# Autodesk Inventor assembly: Base2
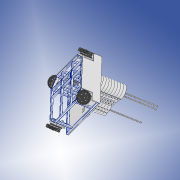
[picture p0: Inventor's stored thumbnail of the model, 180x180]
Saved by Autodesk Inventor 2017 SP1 (Build 210196100, 196)
## iProperties
Created: 2017-06-13
Part Number: Base2
Document SubType Name: Assembly
Designer: zallen
Author: zallen
## Documents named in this file (10)
- C:\Users\Zach\Documents\GitHub\cr-laundry-robot\src\Base\Base.iam
- C:\Users\Zach\Documents\GitHub\cr-laundry-robot\src\Base\Chassis\Chassis.iam
- C:\Users\Zach\Documents\GitHub\cr-laundry-robot\lib\Linear Actuator 450mm\LinearActuator450mm.iam
- C:\Users\Zach\Documents\GitHub\cr-laundry-robot\src\Base\Top Cover.ipt
- C:\Users\Zach\Documents\GitHub\cr-laundry-robot\src\Base\Front Cover.ipt
- C:\Users\Zach\Documents\GitHub\cr-laundry-robot\src\Base\Wheel Assembly\Wheel Assembly.iam
- C:\Users\Zach\Documents\GitHub\cr-laundry-robot\src\Base\Riser Base - Center.ipt
- C:\Users\Zach\Documents\GitHub\cr-laundry-robot\src\Base\Riser Base - Outer.ipt
- C:\Users\Zach\Documents\GitHub\cr-laundry-robot\src\Base\Quick Shaft 12mm x 500mm.ipt
- C:\Users\Zach\Documents\GitHub\cr-laundry-robot\src\Base\Rod End Stop.ipt
## Components (57 placed, 9 different names)
1. Chassis:1 [sub-assembly] — Mate:17, Mate:23, Mate:25, Mate:28, Mate:29, Mate:30, Mate:33, Mate:36, Mate:37, Mate:38, Mate:39, Mate:40, Mate:41, Mate:42, Mate:43, Mate:44, Mate:45, Mate:46, Mate:47, Mate:48, Mate:49, Mate:50, Mate:51, Mate:53, Mate:55
2. LinearActuator450mm:1 [sub-assembly] — Mate:17
3. Top Cover:1 — Mate:23, Mate:24, Mate:26, Mate:27, Mate:31, Mate:32, Mate:34, Mate:52, Mate:54, Mate:57, Mate:159, Mate:161
4. Front Cover:1 — Mate:24, Mate:25, Mate:26, Mate:35
5. Front Cover:2 — Mate:27, Mate:28, Mate:29
6. Front Cover:3 — Mate:33, Mate:34, Mate:35
7. Front Cover:4 — Mate:30, Mate:31, Mate:32
8. Wheel Assembly:1 [sub-assembly] — Mate:36, Mate:37, Mate:38, Mate:39, Mate:40
9. Wheel Assembly:2 [sub-assembly] — Mate:41, Mate:42, Mate:43
10. Wheel Assembly:3 [sub-assembly] — Mate:44, Mate:45, Mate:46
11. Wheel Assembly:4 [sub-assembly] — Mate:47, Mate:48, Mate:49
12. Riser Base - Center:1 — Mate:50, Mate:51, Mate:52, Flush:60, Mate:58, Mate:137, Mate:138
13. Riser Base - Center:2 — Mate:53, Mate:54, Mate:55, Mate:56, Flush:58, Flush:59, Flush:61, Mate:119
14. Riser Base - Outer:1 — Mate:56, Flush:58, Flush:59, Mate:86, Mate:87, Mate:88
15. Riser Base - Outer:2 — Flush:60, Mate:57, Mate:58, Mate:59, Mate:60, Mate:61
16. Riser Base - Outer:3 — Mate:59, Mate:60, Mate:61, Mate:62, Mate:63, Mate:64
17. Riser Base - Outer:4 — Mate:68, Mate:69, Mate:70, Mate:71, Mate:72, Mate:73
18. Riser Base - Outer:5 — Mate:65, Mate:66, Mate:67, Mate:68, Mate:69, Mate:70
19. Riser Base - Outer:6 — Mate:62, Mate:63, Mate:64, Mate:65, Mate:66, Mate:67
20. Riser Base - Outer:7 — Mate:74, Mate:75, Mate:76, Mate:77, Mate:78, Mate:79
21. Riser Base - Outer:8 — Mate:80, Mate:81, Mate:82, Mate:83, Mate:84, Mate:85
22. Riser Base - Outer:9 — Mate:83, Mate:84, Mate:85, Mate:157
23. Riser Base - Outer:10 — Mate:77, Mate:78, Mate:79, Mate:80, Mate:81, Mate:82
24. Riser Base - Outer:11 — Mate:71, Mate:72, Mate:73, Mate:74, Mate:75, Mate:76
25. Riser Base - Outer:12 — Mate:86, Mate:87, Mate:88, Mate:89, Mate:90, Mate:91
26. Riser Base - Outer:13 — Mate:92, Mate:93, Mate:94, Mate:95, Mate:96, Mate:97
27. Riser Base - Outer:14 — Mate:98, Mate:99, Mate:100, Mate:101, Mate:102, Mate:104, Mate:105, Mate:106
28. Riser Base - Outer:15 — Mate:107, Mate:108, Mate:109, Mate:110, Mate:111, Mate:112, Mate:115
29. Riser Base - Outer:16 — Mate:113, Mate:114, Mate:115
30. Riser Base - Outer:17 — Mate:110, Mate:111, Mate:112, Mate:113, Mate:114, Mate:116, Mate:117, Mate:118
31. Riser Base - Outer:18 — Mate:95, Mate:96, Mate:97, Mate:98, Mate:99, Mate:100, Mate:103
32. Riser Base - Outer:19 — Mate:89, Mate:90, Mate:91, Mate:92, Mate:93, Mate:94
33. Riser Base - Outer:20 — Mate:101, Mate:102, Mate:103
34. Riser Base - Outer:21 — Mate:104, Mate:105, Mate:106, Mate:107, Mate:108, Mate:109
35. Riser Base - Outer:22 — Mate:116, Mate:117, Mate:118, Mate:155, Mate:158
36. Riser Base - Center:3 — Mate:120, Mate:121, Mate:122, Mate:123, Mate:124
37. Riser Base - Center:4 — Flush:61, Mate:119, Mate:120, Mate:121
38. Riser Base - Center:5 — Mate:122, Mate:123, Mate:124, Mate:125, Mate:126
39. Riser Base - Center:6 — Mate:129, Mate:130, Mate:131, Mate:132
40. Riser Base - Center:7 — Mate:127, Mate:128, Mate:129, Mate:130
41. Riser Base - Center:8 — Mate:125, Mate:126, Mate:127, Mate:128
42. Riser Base - Center:9 — Mate:131, Mate:132, Mate:133, Mate:134
43. Riser Base - Center:10 — Mate:133, Mate:134, Mate:135, Mate:136
44. Riser Base - Center:11 — Mate:135, Mate:136, Mate:155
45. Riser Base - Center:12 — Mate:137, Mate:138, Mate:139, Mate:140
46. Riser Base - Center:13 — Mate:139, Mate:140, Mate:141, Mate:142
47. Riser Base - Center:14 — Mate:141, Mate:142, Mate:143, Mate:144
48. Riser Base - Center:15 — Mate:143, Mate:144, Mate:145, Mate:146
49. Riser Base - Center:16 — Mate:145, Mate:146, Mate:147, Mate:148
50. Riser Base - Center:17 — Mate:147, Mate:148, Mate:149, Mate:150
51. Riser Base - Center:18 — Mate:149, Mate:150, Mate:151, Mate:152
52. Riser Base - Center:19 — Mate:151, Mate:152, Mate:153, Mate:154
53. Riser Base - Center:20 — Mate:153, Mate:154, Mate:160, Mate:162
54. Quick Shaft 12mm x 500mm:1 — Mate:157, Flush:62, Mate:159
55. Quick Shaft 12mm x 500mm:2 — Mate:158, Flush:62
56. Quick Shaft 12mm x 500mm:3 — Mate:162, Mate:163
57. Rod End Stop:1 — Mate:160, Mate:161, Mate:163
## Relationships (146: Mate 141, Flush 5)
- Mate:17: Chassis:1 ↔ LinearActuator450mm:1
- Mate:23: Chassis:1 ↔ Top Cover:1
- Mate:24: Top Cover:1 ↔ Front Cover:1
- Mate:25: Chassis:1 ↔ Front Cover:1
- Mate:26: Top Cover:1 ↔ Front Cover:1
- Mate:27: Top Cover:1 ↔ Front Cover:2
- Mate:28: Chassis:1 ↔ Front Cover:2
- Mate:29: Chassis:1 ↔ Front Cover:2
- Mate:30: Chassis:1 ↔ Front Cover:4
- Mate:31: Top Cover:1 ↔ Front Cover:4
- Mate:32: Top Cover:1 ↔ Front Cover:4
- Mate:33: Chassis:1 ↔ Front Cover:3
- Mate:34: Top Cover:1 ↔ Front Cover:3
- Mate:35: Front Cover:1 ↔ Front Cover:3
- Mate:36: Chassis:1 ↔ Wheel Assembly:1
- Mate:37: Chassis:1 ↔ Wheel Assembly:1
- Mate:38: Chassis:1 ↔ Wheel Assembly:1
- Mate:39: Chassis:1 ↔ Wheel Assembly:1
- Mate:40: Chassis:1 ↔ Wheel Assembly:1
- Mate:41: Chassis:1 ↔ Wheel Assembly:2
- Mate:42: Chassis:1 ↔ Wheel Assembly:2
- Mate:43: Chassis:1 ↔ Wheel Assembly:2
- Mate:44: Chassis:1 ↔ Wheel Assembly:3
- Mate:45: Chassis:1 ↔ Wheel Assembly:3
- Mate:46: Chassis:1 ↔ Wheel Assembly:3
- Mate:47: Chassis:1 ↔ Wheel Assembly:4
- Mate:48: Chassis:1 ↔ Wheel Assembly:4
- Mate:49: Chassis:1 ↔ Wheel Assembly:4
- Mate:50: Chassis:1 ↔ Riser Base - Center:1
- Mate:51: Chassis:1 ↔ Riser Base - Center:1
- Mate:52: Top Cover:1 ↔ Riser Base - Center:1
- Mate:53: Chassis:1 ↔ Riser Base - Center:2
- Mate:54: Top Cover:1 ↔ Riser Base - Center:2
- Mate:55: Chassis:1 ↔ Riser Base - Center:2
- Mate:56: Riser Base - Center:2 ↔ Riser Base - Outer:1
- Flush:58: Riser Base - Center:2 ↔ Riser Base - Outer:1
- Flush:59: Riser Base - Center:2 ↔ Riser Base - Outer:1
- Flush:60: Riser Base - Center:1 ↔ Riser Base - Outer:2
- Mate:57: Top Cover:1 ↔ Riser Base - Outer:2
- Mate:58: Riser Base - Center:1 ↔ Riser Base - Outer:2
- Mate:59: Riser Base - Outer:2 ↔ Riser Base - Outer:3
- Mate:60: Riser Base - Outer:2 ↔ Riser Base - Outer:3
- Mate:61: Riser Base - Outer:2 ↔ Riser Base - Outer:3
- Mate:62: Riser Base - Outer:3 ↔ Riser Base - Outer:6
- Mate:63: Riser Base - Outer:3 ↔ Riser Base - Outer:6
- Mate:64: Riser Base - Outer:3 ↔ Riser Base - Outer:6
- Mate:65: Riser Base - Outer:5 ↔ Riser Base - Outer:6
- Mate:66: Riser Base - Outer:5 ↔ Riser Base - Outer:6
- Mate:67: Riser Base - Outer:5 ↔ Riser Base - Outer:6
- Mate:68: Riser Base - Outer:4 ↔ Riser Base - Outer:5
- Mate:69: Riser Base - Outer:4 ↔ Riser Base - Outer:5
- Mate:70: Riser Base - Outer:4 ↔ Riser Base - Outer:5
- Mate:71: Riser Base - Outer:4 ↔ Riser Base - Outer:11
- Mate:72: Riser Base - Outer:4 ↔ Riser Base - Outer:11
- Mate:73: Riser Base - Outer:4 ↔ Riser Base - Outer:11
- Mate:74: Riser Base - Outer:7 ↔ Riser Base - Outer:11
- Mate:75: Riser Base - Outer:7 ↔ Riser Base - Outer:11
- Mate:76: Riser Base - Outer:7 ↔ Riser Base - Outer:11
- Mate:77: Riser Base - Outer:7 ↔ Riser Base - Outer:10
- Mate:78: Riser Base - Outer:7 ↔ Riser Base - Outer:10
- Mate:79: Riser Base - Outer:7 ↔ Riser Base - Outer:10
- Mate:80: Riser Base - Outer:8 ↔ Riser Base - Outer:10
- Mate:81: Riser Base - Outer:8 ↔ Riser Base - Outer:10
- Mate:82: Riser Base - Outer:8 ↔ Riser Base - Outer:10
- Mate:83: Riser Base - Outer:8 ↔ Riser Base - Outer:9
- Mate:84: Riser Base - Outer:8 ↔ Riser Base - Outer:9
- Mate:85: Riser Base - Outer:8 ↔ Riser Base - Outer:9
- Mate:86: Riser Base - Outer:1 ↔ Riser Base - Outer:12
- Mate:87: Riser Base - Outer:1 ↔ Riser Base - Outer:12
- Mate:88: Riser Base - Outer:1 ↔ Riser Base - Outer:12
- Mate:89: Riser Base - Outer:12 ↔ Riser Base - Outer:19
- Mate:90: Riser Base - Outer:12 ↔ Riser Base - Outer:19
- Mate:91: Riser Base - Outer:12 ↔ Riser Base - Outer:19
- Mate:92: Riser Base - Outer:13 ↔ Riser Base - Outer:19
- Mate:93: Riser Base - Outer:13 ↔ Riser Base - Outer:19
- Mate:94: Riser Base - Outer:13 ↔ Riser Base - Outer:19
- Mate:95: Riser Base - Outer:13 ↔ Riser Base - Outer:18
- Mate:96: Riser Base - Outer:13 ↔ Riser Base - Outer:18
- Mate:97: Riser Base - Outer:13 ↔ Riser Base - Outer:18
- Mate:98: Riser Base - Outer:14 ↔ Riser Base - Outer:18
- Mate:99: Riser Base - Outer:14 ↔ Riser Base - Outer:18
- Mate:100: Riser Base - Outer:14 ↔ Riser Base - Outer:18
- Mate:101: Riser Base - Outer:14 ↔ Riser Base - Outer:20
- Mate:102: Riser Base - Outer:14 ↔ Riser Base - Outer:20
- Mate:103: Riser Base - Outer:18 ↔ Riser Base - Outer:20
- Mate:104: Riser Base - Outer:14 ↔ Riser Base - Outer:21
- Mate:105: Riser Base - Outer:14 ↔ Riser Base - Outer:21
- Mate:106: Riser Base - Outer:14 ↔ Riser Base - Outer:21
- Mate:107: Riser Base - Outer:15 ↔ Riser Base - Outer:21
- Mate:108: Riser Base - Outer:15 ↔ Riser Base - Outer:21
- Mate:109: Riser Base - Outer:15 ↔ Riser Base - Outer:21
- Mate:110: Riser Base - Outer:15 ↔ Riser Base - Outer:17
- Mate:111: Riser Base - Outer:15 ↔ Riser Base - Outer:17
- Mate:112: Riser Base - Outer:15 ↔ Riser Base - Outer:17
- Mate:113: Riser Base - Outer:16 ↔ Riser Base - Outer:17
- Mate:114: Riser Base - Outer:16 ↔ Riser Base - Outer:17
- Mate:115: Riser Base - Outer:15 ↔ Riser Base - Outer:16
- Mate:116: Riser Base - Outer:17 ↔ Riser Base - Outer:22
- Mate:117: Riser Base - Outer:17 ↔ Riser Base - Outer:22
- Mate:118: Riser Base - Outer:17 ↔ Riser Base - Outer:22
- Flush:61: Riser Base - Center:2 ↔ Riser Base - Center:4
- Mate:119: Riser Base - Center:2 ↔ Riser Base - Center:4
- Mate:120: Riser Base - Center:3 ↔ Riser Base - Center:4
- Mate:121: Riser Base - Center:3 ↔ Riser Base - Center:4
- Mate:122: Riser Base - Center:3 ↔ Riser Base - Center:5
- Mate:123: Riser Base - Center:3 ↔ Riser Base - Center:5
- Mate:124: Riser Base - Center:3 ↔ Riser Base - Center:5
- Mate:125: Riser Base - Center:5 ↔ Riser Base - Center:8
- Mate:126: Riser Base - Center:5 ↔ Riser Base - Center:8
- Mate:127: Riser Base - Center:7 ↔ Riser Base - Center:8
- Mate:128: Riser Base - Center:7 ↔ Riser Base - Center:8
- Mate:129: Riser Base - Center:6 ↔ Riser Base - Center:7
- Mate:130: Riser Base - Center:6 ↔ Riser Base - Center:7
- Mate:131: Riser Base - Center:6 ↔ Riser Base - Center:9
- Mate:132: Riser Base - Center:6 ↔ Riser Base - Center:9
- Mate:133: Riser Base - Center:9 ↔ Riser Base - Center:10
- Mate:134: Riser Base - Center:9 ↔ Riser Base - Center:10
- Mate:135: Riser Base - Center:10 ↔ Riser Base - Center:11
- Mate:136: Riser Base - Center:10 ↔ Riser Base - Center:11
- Mate:137: Riser Base - Center:1 ↔ Riser Base - Center:12
- Mate:138: Riser Base - Center:1 ↔ Riser Base - Center:12
- Mate:139: Riser Base - Center:12 ↔ Riser Base - Center:13
- Mate:140: Riser Base - Center:12 ↔ Riser Base - Center:13
- Mate:141: Riser Base - Center:13 ↔ Riser Base - Center:14
- Mate:142: Riser Base - Center:13 ↔ Riser Base - Center:14
- Mate:143: Riser Base - Center:14 ↔ Riser Base - Center:15
- Mate:144: Riser Base - Center:14 ↔ Riser Base - Center:15
- Mate:145: Riser Base - Center:15 ↔ Riser Base - Center:16
- Mate:146: Riser Base - Center:15 ↔ Riser Base - Center:16
- Mate:147: Riser Base - Center:16 ↔ Riser Base - Center:17
- Mate:148: Riser Base - Center:16 ↔ Riser Base - Center:17
- Mate:149: Riser Base - Center:17 ↔ Riser Base - Center:18
- Mate:150: Riser Base - Center:17 ↔ Riser Base - Center:18
- Mate:151: Riser Base - Center:18 ↔ Riser Base - Center:19
- Mate:152: Riser Base - Center:18 ↔ Riser Base - Center:19
- Mate:153: Riser Base - Center:19 ↔ Riser Base - Center:20
- Mate:154: Riser Base - Center:19 ↔ Riser Base - Center:20
- Mate:155: Riser Base - Outer:22 ↔ Riser Base - Center:11
- Mate:157: Riser Base - Outer:9 ↔ Quick Shaft 12mm x 500mm:1
- Mate:158: Riser Base - Outer:22 ↔ Quick Shaft 12mm x 500mm:2
- Flush:62: Quick Shaft 12mm x 500mm:1 ↔ Quick Shaft 12mm x 500mm:2
- Mate:159: Top Cover:1 ↔ Quick Shaft 12mm x 500mm:1
- Mate:160: Riser Base - Center:20 ↔ Rod End Stop:1
- Mate:161: Top Cover:1 ↔ Rod End Stop:1
- Mate:162: Riser Base - Center:20 ↔ Quick Shaft 12mm x 500mm:3
- Mate:163: Quick Shaft 12mm x 500mm:3 ↔ Rod End Stop:1
